# Autodesk Inventor assembly: robotic_arm
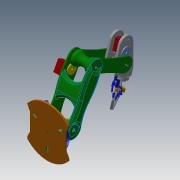
[picture p0: Inventor's stored thumbnail of the model, 180x180]
Saved by Autodesk Inventor 2013 (Build 170138000, 138)
## iProperties
Created: 2013-05-11
Part Number: robotic_arm
Document SubType Name: Assembly
Designer: idle-rug
Author: idle-rug
## Documents named in this file (27)
- C:\Users\Petr\Documents\Inventor\robotic arm\rameno\robotic_arm.iam
- C:\Users\Petr\Documents\Inventor\robotic arm\rameno\standart_servo.ipt
- C:\Users\Petr\Documents\Inventor\robotic arm\rameno\rameno(a)nahore.ipt
- C:\Users\Petr\Documents\Inventor\robotic arm\rameno\rameno(b)nahore.ipt
- C:\Users\Petr\Documents\Inventor\robotic arm\rameno\kolecko_servo(3).ipt
- C:\Users\Petr\Documents\Inventor\robotic arm\rameno\kolecko_rameno(2).ipt
- C:\Users\Petr\Documents\Inventor\robotic arm\rameno\packa_strana(a).ipt
- C:\Users\Petr\Documents\Inventor\robotic arm\rameno\packa_strana(b).ipt
- C:\Users\Petr\Documents\Inventor\robotic arm\rameno\kolecko_rameno(3).ipt
- C:\Users\Petr\Documents\Inventor\robotic arm\rameno\rameno(b)dole.ipt
- C:\Users\Petr\Documents\Inventor\robotic arm\rameno\rameno(a)dole.ipt
- C:\Users\Petr\Documents\Inventor\robotic arm\rameno\kolecko_servo(2).ipt
- C:\Users\Petr\Documents\Inventor\robotic arm\rameno\servo_paka_dolu.ipt
- C:\Users\Petr\Documents\Inventor\robotic arm\rameno\otocni_kruh(svrchni).ipt
- C:\Users\Petr\Documents\Inventor\robotic arm\micro_servo.ipt
- C:\Users\Petr\Documents\Inventor\robotic arm\rameno\otaceni_packy_microservo.ipt
- C:\Users\Petr\Documents\Inventor\robotic arm\ruka_backup.iam
- C:\Users\Petr\Documents\Inventor\robotic arm\rameno\hridelka_packa.ipt
- C:\Users\Petr\Documents\Inventor\robotic arm\rameno\hridel1.ipt
- C:\Users\Petr\Documents\Inventor\robotic arm\rameno\hridel2.ipt
- C:\Users\Petr\Documents\Inventor\robotic arm\rameno\vystuha_hridel_nahore.ipt
- C:\Users\Petr\Documents\Inventor\robotic arm\rameno\stojan2.ipt
- C:\Users\Petr\Documents\Inventor\robotic arm\rameno\otaceni_ramene_motor.ipt
- C:\Users\Petr\Documents\Inventor\robotic arm\rameno\ozubene_kolecko_otaceni_ramene_male.ipt
- C:\Users\Petr\Documents\Inventor\robotic arm\rameno\deska-pod_otocny kruh.ipt
- C:\Users\Petr\Documents\Inventor\robotic arm\rameno\velke_kolecko_rameno_otaceni.ipt
- C:\Users\Petr\Documents\Inventor\robotic arm\rameno\valecky_na_otocny_kruh.ipt
## Components (32 placed, 26 different names)
1. packa_strana(a):1 — Mate:53, Mate:55, Mate:56, Mate:57, Mate:58, Mate:59, Mate:128, Mate:196
2. packa_strana(b):1 — Flush:1, Mate:59, Mate:60, Mate:109, Mate:114, Mate:115, Mate:124, Mate:214
3. standart_servo:3 — Mate:53, Mate:55, Mate:56, Mate:57, Mate:58, Flush:1, Mate:60, Mate:61, Mate:62
4. kolecko_servo(3):1 — Mate:61, Mate:62, Flush:2, Mate:196
5. kolecko_rameno(3):1 — Flush:2, Mate:128, Mate:152, Mate:156, Mate:215
6. rameno(b)nahore:1 — Mate:72, Mate:73, Mate:124, Mate:135, Mate:160, Mate:162, Mate:173
7. kolecko_rameno(2):1 — Mate:72, Mate:73, Mate:135, Mate:148, Mate:149
8. rameno(b)dole:1 — Mate:77, Mate:78, Mate:79, Mate:87, Mate:88, Mate:117, Mate:132, Mate:133, Mate:134, Mate:148, Mate:149, Mate:170, Mate:183
9. standart_servo:4 — Mate:77, Mate:78, Mate:79, Mate:80, Mate:81, Mate:132, Mate:133, Mate:134
10. kolecko_servo(2):1 — Mate:80, Mate:81
11. servo_paka_dolu:1 — Mate:87, Mate:88, Mate:90, Mate:117, Mate:118, Mate:119
12. standart_servo:5 — Mate:90, Mate:118, Mate:119, Mate:186, Mate:187, Mate:188, Mate:189
13. otocni_kruh(svrchni):1 — Mate:174, Mate:175, Mate:177, Mate:178, Mate:179, Mate:180, Mate:181, Mate:182, Mate:186, Mate:187, Mate:188, Mate:189, Mate:192, Mate:193, Mate:194, Mate:200
14. micro_servo:1 — Mate:103, Mate:104, Mate:109, Mate:112, Mate:114, Mate:115
15. otaceni_packy_microservo:1 — Mate:103, Mate:104, Mate:111, Mate:198
16. ruka_backup:1 [sub-assembly] — Mate:199, Mate:213, Mate:214
17. hridelka_packa:1 — Mate:111, Mate:112, Mate:198, Mate:199, Mate:213
18. rameno(a)dole:3 — Mate:150, Flush:3, Flush:4, Mate:155, Mate:164, Mate:167, Mate:172
19. hridel1:1 — Mate:150, Flush:3, Mate:154, Mate:163, Mate:172, Mate:173
20. hridel1:2 — Flush:4, Mate:166, Mate:167, Mate:183
21. hridel2:1 — Mate:153, Mate:156, Flush:5, Mate:160
22. rameno(a)nahore:2 — Mate:152, Mate:153, Mate:154, Mate:155, Flush:5, Mate:161, Mate:215
23. vystuha_hridel_nahore:2 — Mate:161, Mate:162, Mate:163
24. stojan2:1 — Mate:164, Mate:166, Mate:175, Mate:177, Mate:178, Mate:180
25. stojan2:2 — Mate:170, Mate:174, Mate:179, Mate:181, Mate:182
26. otaceni_ramene_motor:1 — Mate:191, Mate:192, Mate:194
27. ozubene_kolecko_otaceni_ramene_male:1 — Mate:191, Mate:193, Flush:6
28. deska-pod_otocny kruh:1 — Mate:200, Mate:202, Mate:203, Mate:204, Mate:205, Mate:206, Mate:207, Mate:208, Mate:209, Mate:210, Mate:211, Mate:212
29. velke_kolecko_rameno_otaceni:1 — Mate:202, Flush:6, Mate:209, Mate:210
30. valecky_na_otocny_kruh:1 — Mate:203, Mate:204
31. valecky_na_otocny_kruh:2 — Mate:205, Mate:206
32. valecky_na_otocny_kruh:3 — Mate:207, Mate:208
## Relationships (94: Mate 88, Flush 6)
- Mate:53: packa_strana(a):1 ↔ standart_servo:3
- Mate:55: packa_strana(a):1 ↔ standart_servo:3
- Mate:56: packa_strana(a):1 ↔ standart_servo:3
- Mate:57: packa_strana(a):1 ↔ standart_servo:3
- Mate:58: packa_strana(a):1 ↔ standart_servo:3
- Flush:1: packa_strana(b):1 ↔ standart_servo:3
- Mate:59: packa_strana(a):1 ↔ packa_strana(b):1
- Mate:60: packa_strana(b):1 ↔ standart_servo:3
- Mate:61: standart_servo:3 ↔ kolecko_servo(3):1
- Mate:62: standart_servo:3 ↔ kolecko_servo(3):1
- Flush:2: kolecko_servo(3):1 ↔ kolecko_rameno(3):1
- Mate:72: rameno(b)nahore:1 ↔ kolecko_rameno(2):1
- Mate:73: rameno(b)nahore:1 ↔ kolecko_rameno(2):1
- Mate:77: rameno(b)dole:1 ↔ standart_servo:4
- Mate:78: rameno(b)dole:1 ↔ standart_servo:4
- Mate:79: rameno(b)dole:1 ↔ standart_servo:4
- Mate:80: standart_servo:4 ↔ kolecko_servo(2):1
- Mate:81: standart_servo:4 ↔ kolecko_servo(2):1
- Mate:87: rameno(b)dole:1 ↔ servo_paka_dolu:1
- Mate:88: rameno(b)dole:1 ↔ servo_paka_dolu:1
- Mate:90: servo_paka_dolu:1 ↔ standart_servo:5
- Mate:103: micro_servo:1 ↔ otaceni_packy_microservo:1
- Mate:104: micro_servo:1 ↔ otaceni_packy_microservo:1
- Mate:109: packa_strana(b):1 ↔ micro_servo:1
- Mate:111: otaceni_packy_microservo:1 ↔ hridelka_packa:1
- Mate:112: micro_servo:1 ↔ hridelka_packa:1
- Mate:114: packa_strana(b):1 ↔ micro_servo:1
- Mate:115: packa_strana(b):1 ↔ micro_servo:1
- Mate:117 (2 mm): rameno(b)dole:1 ↔ servo_paka_dolu:1
- Mate:118: servo_paka_dolu:1 ↔ standart_servo:5
- Mate:119: servo_paka_dolu:1 ↔ standart_servo:5
- Mate:124 (2 mm): packa_strana(b):1 ↔ rameno(b)nahore:1
- Mate:128: packa_strana(a):1 ↔ kolecko_rameno(3):1
- Mate:132: rameno(b)dole:1 ↔ standart_servo:4
- Mate:133: rameno(b)dole:1 ↔ standart_servo:4
- Mate:134: rameno(b)dole:1 ↔ standart_servo:4
- Mate:135 (2 mm): rameno(b)nahore:1 ↔ kolecko_rameno(2):1
- Mate:148: kolecko_rameno(2):1 ↔ rameno(b)dole:1
- Mate:149: kolecko_rameno(2):1 ↔ rameno(b)dole:1
- Mate:150: rameno(a)dole:3 ↔ hridel1:1
- Flush:3: rameno(a)dole:3 ↔ hridel1:1
- Flush:4: rameno(a)dole:3 ↔ hridel1:2
- Mate:152 (2 mm): kolecko_rameno(3):1 ↔ rameno(a)nahore:2
- Mate:153: hridel2:1 ↔ rameno(a)nahore:2
- Mate:154: hridel1:1 ↔ rameno(a)nahore:2
- Mate:155 (2 mm): rameno(a)dole:3 ↔ rameno(a)nahore:2
- Mate:156: kolecko_rameno(3):1 ↔ hridel2:1
- Flush:5: hridel2:1 ↔ rameno(a)nahore:2
- Mate:160: rameno(b)nahore:1 ↔ hridel2:1
- Mate:161: rameno(a)nahore:2 ↔ vystuha_hridel_nahore:2
- Mate:162: rameno(b)nahore:1 ↔ vystuha_hridel_nahore:2
- Mate:163: hridel1:1 ↔ vystuha_hridel_nahore:2
- Mate:164 (2 mm): rameno(a)dole:3 ↔ stojan2:1
- Mate:166: hridel1:2 ↔ stojan2:1
- Mate:167: rameno(a)dole:3 ↔ hridel1:2
- Mate:170 (2 mm): rameno(b)dole:1 ↔ stojan2:2
- Mate:172: rameno(a)dole:3 ↔ hridel1:1
- Mate:173: rameno(b)nahore:1 ↔ hridel1:1
- Mate:174: otocni_kruh(svrchni):1 ↔ stojan2:2
- Mate:175: otocni_kruh(svrchni):1 ↔ stojan2:1
- Mate:177: otocni_kruh(svrchni):1 ↔ stojan2:1
- Mate:178: otocni_kruh(svrchni):1 ↔ stojan2:1
- Mate:179: otocni_kruh(svrchni):1 ↔ stojan2:2
- Mate:180: otocni_kruh(svrchni):1 ↔ stojan2:1
- Mate:181: otocni_kruh(svrchni):1 ↔ stojan2:2
- Mate:182: otocni_kruh(svrchni):1 ↔ stojan2:2
- Mate:183: rameno(b)dole:1 ↔ hridel1:2
- Mate:186: standart_servo:5 ↔ otocni_kruh(svrchni):1
- Mate:187: standart_servo:5 ↔ otocni_kruh(svrchni):1
- Mate:188: standart_servo:5 ↔ otocni_kruh(svrchni):1
- Mate:189: standart_servo:5 ↔ otocni_kruh(svrchni):1
- Mate:191: otaceni_ramene_motor:1 ↔ ozubene_kolecko_otaceni_ramene_male:1
- Mate:192: otocni_kruh(svrchni):1 ↔ otaceni_ramene_motor:1
- Mate:193 (2 mm): otocni_kruh(svrchni):1 ↔ ozubene_kolecko_otaceni_ramene_male:1
- Mate:194: otocni_kruh(svrchni):1 ↔ otaceni_ramene_motor:1
- Mate:196 (2 mm): packa_strana(a):1 ↔ kolecko_servo(3):1
- Mate:198: otaceni_packy_microservo:1 ↔ hridelka_packa:1
- Mate:199: ruka_backup:1 ↔ hridelka_packa:1
- Mate:200: otocni_kruh(svrchni):1 ↔ deska-pod_otocny kruh:1
- Mate:202: deska-pod_otocny kruh:1 ↔ velke_kolecko_rameno_otaceni:1
- Mate:203: deska-pod_otocny kruh:1 ↔ valecky_na_otocny_kruh:1
- Mate:204 (0.25 mm): deska-pod_otocny kruh:1 ↔ valecky_na_otocny_kruh:1
- Mate:205: deska-pod_otocny kruh:1 ↔ valecky_na_otocny_kruh:2
- Mate:206 (0.25 mm): deska-pod_otocny kruh:1 ↔ valecky_na_otocny_kruh:2
- Mate:207: deska-pod_otocny kruh:1 ↔ valecky_na_otocny_kruh:3
- Mate:208 (0.25 mm): deska-pod_otocny kruh:1 ↔ valecky_na_otocny_kruh:3
- Flush:6: ozubene_kolecko_otaceni_ramene_male:1 ↔ velke_kolecko_rameno_otaceni:1
- Mate:209: deska-pod_otocny kruh:1 ↔ velke_kolecko_rameno_otaceni:1
- Mate:210 (2 mm): deska-pod_otocny kruh:1 ↔ velke_kolecko_rameno_otaceni:1
- Mate:211: deska-pod_otocny kruh:1
- Mate:212: deska-pod_otocny kruh:1
- Mate:213: ruka_backup:1 ↔ hridelka_packa:1
- Mate:214 (2 mm): packa_strana(b):1 ↔ ruka_backup:1
- Mate:215: kolecko_rameno(3):1 ↔ rameno(a)nahore:2
